# Autodesk Inventor assembly: joint_meteor
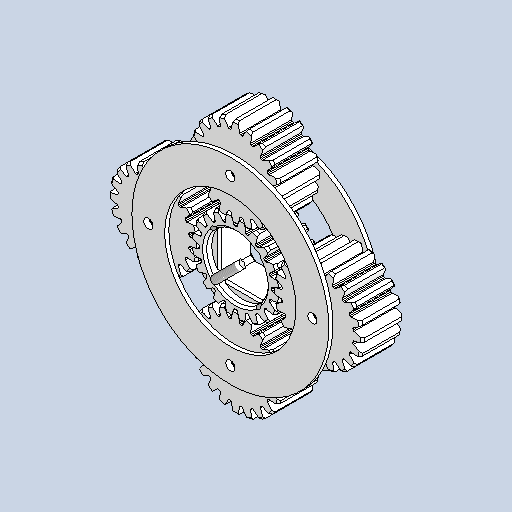
[picture p0: Inventor's stored thumbnail of the model, 512x512]
Saved by Autodesk Inventor 2025.3 (Build 293356030, 356C)
## iProperties
Created: 2025-09-07
Part Number: joint_meteor
Document SubType Name: Assembly
Designer: MSI
Mass: 150.332 g
Surface Area: 636.036 cm^2
Volume: 125.548 cm^3
Density: 1.19741 g/cm^3
Author: MSI
## Documents named in this file (8)
- C:\Users\MSI\Desktop\Project\3. 로봇팔\Robot Arm Model\joint3\joint3_meteor.iam
- C:\Users\MSI\Desktop\Project\3. 로봇팔\Robot Arm Model\joint3\joint3_meteor\디자인 액셀러레이터\스퍼 기어1.iam
- C:\Users\MSI\Desktop\Project\3. 로봇팔\Robot Arm Model\joint3\joint3_meteor\디자인 액셀러레이터\스퍼 기어2.iam
- C:\Users\MSI\Desktop\Project\3. 로봇팔\Robot Arm Model\joint3\joint3_meteor\디자인 액셀러레이터\스퍼 기어3.iam
- C:\Users\MSI\Desktop\Project\3. 로봇팔\Robot Arm Model\joint3\joint3_carrier.ipt
- C:\Users\MSI\Desktop\Project\3. 로봇팔\Robot Arm Model\joint3\joint3_asix3.ipt
- C:\Users\MSI\Desktop\Project\3. 로봇팔\Robot Arm Model\joint3\C-E678ZZ_Inventor\C-E678ZZ.ipt
- C:\Users\MSI\Desktop\Project\3. 로봇팔\Robot Arm Model\joint3\Robot_Arm_Parameter.xlsx
## Components (20 placed, 4 different names)
1. 스퍼 기어:1 [sub-assembly] — 메이트:1, 각도:1, 플러쉬:1, 메이트:4, 플러쉬:2, 플러쉬:6, 메이트:5
2. 스퍼 기어:2 [sub-assembly] — 메이트:1, 각도:1, 메이트:3, 플러쉬:2, 메이트:7, 메이트:6
3. joint3_carrier:1 — 삽입:1, 삽입:2
4. joint3_carrier:2 — 삽입:3, 삽입:4
5. 스퍼 기어:3 [sub-assembly] — 플러쉬:1, 플러쉬:6, 메이트:5, 메이트:6, 삽입:5, 삽입:6, 삽입:7
6. joint3_asix3:1 — 삽입:5
7. C-E678ZZ:1 — 삽입:6
8. C-E678ZZ:2 — 삽입:7
9. 스퍼 기어:4 [sub-assembly] — 삽입:1, 삽입:3
10. joint3_asix3:2
11. C-E678ZZ:3
12. C-E678ZZ:6
13. 스퍼 기어:5 [sub-assembly]
14. joint3_asix3:3
15. C-E678ZZ:4
16. C-E678ZZ:7
17. 스퍼 기어:6 [sub-assembly] — 삽입:2, 삽입:4
18. joint3_asix3:4
19. C-E678ZZ:5
20. C-E678ZZ:8
## Component patterns: (4 elements, first: 스퍼 기어:3 + joint3_asix3:1 + C-E678ZZ:1 + C-E678ZZ:2)
## Relationships (17: Insert 7, Mate 6, Flush 3, Angle 1)
- 메이트:1 [Mate]: 스퍼 기어:1 ↔ 스퍼 기어:2
- 각도:1 [Angle] (45 deg): 스퍼 기어:1 ↔ 스퍼 기어:2
- 플러쉬:1 [Flush]: 스퍼 기어:1 ↔ 스퍼 기어:3
- 메이트:3 [Mate]: 스퍼 기어:2
- 메이트:4 [Mate]: 스퍼 기어:1
- 플러쉬:2 [Flush]: 스퍼 기어:1 ↔ 스퍼 기어:2
- 플러쉬:6 [Flush]: 스퍼 기어:1 ↔ 스퍼 기어:3
- 메이트:5 [Mate] (40 mm): 스퍼 기어:1 ↔ 스퍼 기어:3
- 메이트:6 [Mate]: 스퍼 기어:2 ↔ 스퍼 기어:3
- 메이트:7 [Mate]: 스퍼 기어:2
- 삽입:1 [Insert]: joint3_carrier:1 ↔ 스퍼 기어:4
- 삽입:2 [Insert]: joint3_carrier:1 ↔ 스퍼 기어:6
- 삽입:3 [Insert]: joint3_carrier:2 ↔ 스퍼 기어:4
- 삽입:4 [Insert]: joint3_carrier:2 ↔ 스퍼 기어:6
- 삽입:5 [Insert]: 스퍼 기어:3 ↔ joint3_asix3:1
- 삽입:6 [Insert]: 스퍼 기어:3 ↔ C-E678ZZ:1
- 삽입:7 [Insert]: 스퍼 기어:3 ↔ C-E678ZZ:2
## Named parameters: joint4_belt_centor = 157.367 mm, joint4_axis2_L = 58.803 mm, joint4_axis2_b1 = 35 mm, joint4_axis2_b2 = 10 mm, joint4_axis2_d = 19 mm, joint4_miter_m = 2 mm, joint4_miter_a = 20 deg, joint4_miter_z = 79 mm, joint4_miter_b = 6.90139 mm, joint4_axis3_L = 23.5 mm, joint4_axis3_d1 = 30 mm, joint4_axis3_d2 = 50 mm, joint3_belt_centor = 157.367 mm, joint3_axis2_L = 63.75 mm, joint3_axis2_b1 = 38 mm, joint3_axis2_d = 29 mm, joint3_planetary_m = 2 mm, joint3_planetary_a = 20 deg, joint3_planetary_np = 4 mm, joint3_sun_z = 20 mm, joint3_sun_b = 19 mm, joint3_planet_z = 20 mm, joint3_planet_b = 19 mm, joint3_ring_z = 60 mm, joint3_ring_b = 18 mm, joint3_axis3_L = 20 mm, joint3_axis3_d = 29 mm, joint3_miter_m = 4 mm, joint3_miter_a = 20 deg, joint3_miter_z = 28 mm, joint3_miter_b = 25.07657 mm, joint3_axis4_L = 43.706 mm, joint3_axis4_d1 = 30 mm, joint3_axis4_d2 = 50 mm, joint3_miter_z1 = 26 mm, joint3_miter_z2 = 39 mm
